# Autodesk Inventor assembly: Circ case assembly
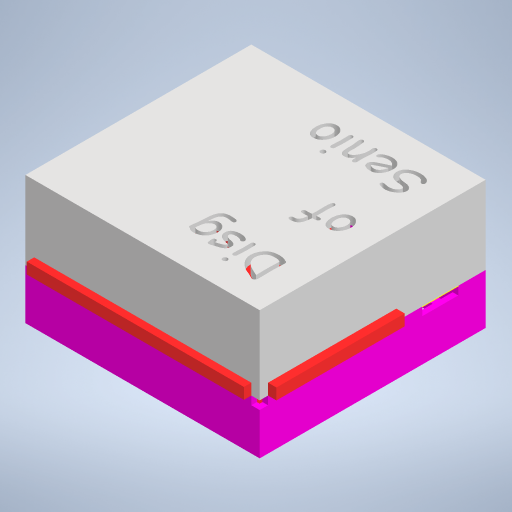
[picture p0: Inventor's stored thumbnail of the model, 512x512]
Saved by Autodesk Inventor 2023 (Build 270158000, 158)
## iProperties
Created: 2022-04-19
Part Number: Circ case assembly
Document SubType Name: Assembly
Designer: cooki
Author: cooki
## Documents named in this file (4)
- C:\Users\cooki\Desktop\Classes\Senior design\Circ case\Circ case assembly.iam
- C:\Users\cooki\Desktop\Classes\Senior design\Circ case\board.ipt
- C:\Users\cooki\Desktop\Classes\Senior design\Circ case\top.ipt
- C:\Users\cooki\Desktop\Classes\Senior design\Circ case\bottom.ipt
## Components (3 placed, 3 different names)
1. board:1 — Flush:1
2. top:1 — Flush:1, Flush:2
3. bottom:1 — Flush:2
## Relationships (2: Flush 2)
- Flush:1: board:1 ↔ top:1
- Flush:2: top:1 ↔ bottom:1
